# Autodesk Inventor assembly: 3d pt end eff
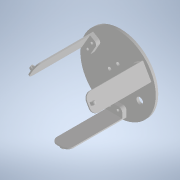
[picture p0: Inventor's stored thumbnail of the model, 180x180]
Saved by Autodesk Inventor 2021 (Build 250183000, 183)
## iProperties
Created: 2021-03-27
Part Number: 3d pt end eff
Document SubType Name: Assembly
Designer: ASUS
Author: ASUS
## Documents named in this file (3)
- E:\borewell rescuebot\pll manipulator files\sps manipulator\3d pt end eff.iam
- E:\borewell rescuebot\pll manipulator files\sps manipulator\base-3dp.ipt
- E:\borewell rescuebot\pll manipulator files\sps manipulator\arms-3dp.ipt
## Components (4 placed, 2 different names)
1. base-3dp:1 — Mate:1, Mate:2, Mate:3
2. arms-3dp:1 — Mate:1, Mate:2, Mate:3
3. arms-3dp:2
4. arms-3dp:3
## Component patterns: (3 elements, first: arms-3dp:1)
## Relationships (3: Mate 3)
- Mate:1: base-3dp:1 ↔ arms-3dp:1
- Mate:2: base-3dp:1 ↔ arms-3dp:1
- Mate:3: base-3dp:1 ↔ arms-3dp:1
